# Autodesk Inventor assembly: OBG-Unterbau
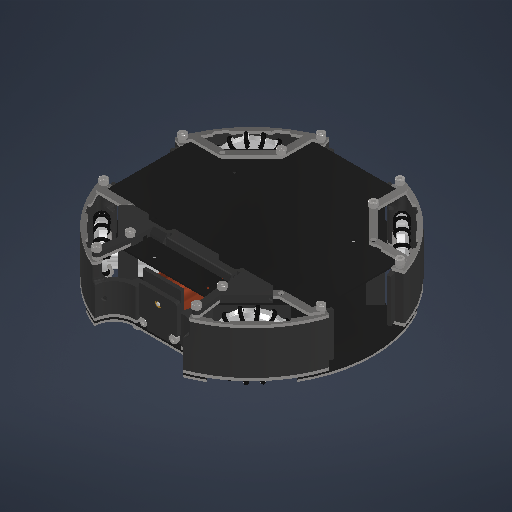
[picture p0: Inventor's stored thumbnail of the model, 512x512]
Saved by Autodesk Inventor 2025.2 (Build 292293000, 293)
## iProperties
Created: 2025-03-27
Part Number: OBG-Unterbau
Document SubType Name: Assembly
Designer: Faabs
Author: Faabs
## Documents named in this file (12)
- C:\Users\Faabs\Desktop\HBG v2023\OBG\Unterbau\OBG-Unterbau.iam
- C:\Users\Faabs\Desktop\HBG v2023\Platinen\Bodenplatine.ipt
- C:\Users\Faabs\Desktop\HBG v2023\UBG\Antrieb\UBG-Antrieb_VR.iam
- C:\Users\Faabs\Desktop\HBG v2023\UBG\Antrieb\UBG-Antrieb_VL.iam
- C:\Users\Faabs\Desktop\HBG v2023\UBG\Antrieb\UBG-Antrieb_HL.iam
- C:\Users\Faabs\Desktop\HBG v2023\UBG\Antrieb\UBG-Antrieb_HR.iam
- C:\Users\Faabs\Desktop\HBG v2023\UBG\Schuss\UBG-Schuss.iam
- C:\Users\Faabs\Desktop\HBG v2023\OBG\Unterbau\Bodenplatinenring.ipt
- C:\Users\Faabs\Desktop\HBG v2023\Platinen\Hauptplatine.ipt
- C:\Users\Faabs\Desktop\HBG v2023\UBG\Schutz\UBG-Schutz.iam
- C:\Users\Faabs\Desktop\HBG v2023\Verbindungselemente\DIN 912\DIN 912 - M3 x 0,5 x 6 x 4,75.ipt
- C:\Users\Faabs\Desktop\HBG v2023\OBG\Unterbau\Dribblerhalterung\Dribblerhalterung\Dribblerhalterung.ipt
## Components (28 placed, 11 different names)
1. UBG-Antrieb_VR:1 [sub-assembly] — Passend:2, Passend:3, Passend:16
2. UBG-Antrieb_VL:1 [sub-assembly] — Passend:4, Passend:5, Passend:15, Passend:20
3. UBG-Antrieb_HL:1 [sub-assembly] — Passend:6, Passend:7, Passend:8, Passend:22
4. UBG-Antrieb_HR:1 [sub-assembly] — Passend:9, Passend:10, Passend:11, Passend:21
5. UBG-Schuss:1 [sub-assembly] — Passend:12, Passend:13, Passend:14, Passend:15, Passend:16
6. UBG-Schutz:1 [sub-assembly] — Passend:23, Passend:24, Passend:25, Einfügen:1, Einfügen:2, Passend:26, Passend:27, Passend:28
7. Bodenplatine:1 — Passend:1, Fluchtend:1, Fluchtend:2, Passend:2, Passend:3, Passend:4, Passend:5, Passend:6, Passend:7, Passend:8, Passend:9, Passend:10, Passend:11, Passend:12, Passend:13, Passend:14, Passend:17, Passend:18, Passend:19, Passend:23, Passend:24, Passend:25
8. Hauptplatine:1 — Passend:20, Passend:21, Passend:22
9. Bodenplatinenring:1 — Passend:17, Passend:18, Passend:19, Einfügen:3, Einfügen:4, Einfügen:5, Einfügen:6, Einfügen:7, Einfügen:8, Einfügen:9, Einfügen:10, Einfügen:11, Einfügen:12, Einfügen:13, Einfügen:14
10. Dribblerhalterung:1 — Passend:26, Passend:27, Passend:28, Einfügen:15, Einfügen:16, Einfügen:17, Einfügen:18
11. DIN 912 - ersetzt durch DIN EN ISO 4762 M3 x 6:18 — Einfügen:17
12. DIN 912 - ersetzt durch DIN EN ISO 4762 M3 x 6:17 — Einfügen:18
13. DIN 912 - ersetzt durch DIN EN ISO 4762 M3 x 6:16 — Einfügen:15
14. DIN 912 - ersetzt durch DIN EN ISO 4762 M3 x 6:15 — Einfügen:16
15. DIN 912 - ersetzt durch DIN EN ISO 4762 M3 x 6:1 — Einfügen:1
16. DIN 912 - ersetzt durch DIN EN ISO 4762 M3 x 6:2 — Einfügen:2
17. DIN 912 - ersetzt durch DIN EN ISO 4762 M3 x 6:3 — Einfügen:5
18. DIN 912 - ersetzt durch DIN EN ISO 4762 M3 x 6:4 — Einfügen:6
19. DIN 912 - ersetzt durch DIN EN ISO 4762 M3 x 6:5 — Einfügen:3
20. DIN 912 - ersetzt durch DIN EN ISO 4762 M3 x 6:6 — Einfügen:4
21. DIN 912 - ersetzt durch DIN EN ISO 4762 M3 x 6:7 — Einfügen:14
22. DIN 912 - ersetzt durch DIN EN ISO 4762 M3 x 6:8 — Einfügen:13
23. DIN 912 - ersetzt durch DIN EN ISO 4762 M3 x 6:9 — Einfügen:12
24. DIN 912 - ersetzt durch DIN EN ISO 4762 M3 x 6:10 — Einfügen:11
25. DIN 912 - ersetzt durch DIN EN ISO 4762 M3 x 6:11 — Einfügen:10
26. DIN 912 - ersetzt durch DIN EN ISO 4762 M3 x 6:12 — Einfügen:9
27. DIN 912 - ersetzt durch DIN EN ISO 4762 M3 x 6:13 — Einfügen:8
28. DIN 912 - ersetzt durch DIN EN ISO 4762 M3 x 6:14 — Einfügen:7
## Relationships (48: Mate 28, Insert 18, Flush 2)
- Passend:1 [Mate]: Bodenplatine:1
- Fluchtend:1 [Flush]: Bodenplatine:1
- Fluchtend:2 [Flush]: Bodenplatine:1
- Passend:2 [Mate]: UBG-Antrieb_VR:1 ↔ Bodenplatine:1
- Passend:3 [Mate]: UBG-Antrieb_VR:1 ↔ Bodenplatine:1
- Passend:4 [Mate]: UBG-Antrieb_VL:1 ↔ Bodenplatine:1
- Passend:5 [Mate]: UBG-Antrieb_VL:1 ↔ Bodenplatine:1
- Passend:6 [Mate]: UBG-Antrieb_HL:1 ↔ Bodenplatine:1
- Passend:7 [Mate]: UBG-Antrieb_HL:1 ↔ Bodenplatine:1
- Passend:8 [Mate]: UBG-Antrieb_HL:1 ↔ Bodenplatine:1
- Passend:9 [Mate]: UBG-Antrieb_HR:1 ↔ Bodenplatine:1
- Passend:10 [Mate]: UBG-Antrieb_HR:1 ↔ Bodenplatine:1
- Passend:11 [Mate]: UBG-Antrieb_HR:1 ↔ Bodenplatine:1
- Passend:12 [Mate]: UBG-Schuss:1 ↔ Bodenplatine:1
- Passend:13 [Mate]: UBG-Schuss:1 ↔ Bodenplatine:1
- Passend:14 [Mate]: UBG-Schuss:1 ↔ Bodenplatine:1
- Passend:15 [Mate]: UBG-Antrieb_VL:1 ↔ UBG-Schuss:1
- Passend:16 [Mate]: UBG-Antrieb_VR:1 ↔ UBG-Schuss:1
- Passend:17 [Mate]: Bodenplatine:1 ↔ Bodenplatinenring:1
- Passend:18 [Mate]: Bodenplatine:1 ↔ Bodenplatinenring:1
- Passend:19 [Mate]: Bodenplatine:1 ↔ Bodenplatinenring:1
- Passend:20 [Mate]: UBG-Antrieb_VL:1 ↔ Hauptplatine:1
- Passend:21 [Mate]: UBG-Antrieb_HR:1 ↔ Hauptplatine:1
- Passend:22 [Mate]: UBG-Antrieb_HL:1 ↔ Hauptplatine:1
- Passend:23 [Mate]: UBG-Schutz:1 ↔ Bodenplatine:1
- Passend:24 [Mate]: UBG-Schutz:1 ↔ Bodenplatine:1
- Passend:25 [Mate]: UBG-Schutz:1 ↔ Bodenplatine:1
- Einfügen:1 [Insert]: UBG-Schutz:1 ↔ DIN 912 - ersetzt durch DIN EN ISO 4762 M3 x 6:1
- Einfügen:2 [Insert]: UBG-Schutz:1 ↔ DIN 912 - ersetzt durch DIN EN ISO 4762 M3 x 6:2
- Einfügen:3 [Insert]: Bodenplatinenring:1 ↔ DIN 912 - ersetzt durch DIN EN ISO 4762 M3 x 6:5
- Einfügen:4 [Insert]: Bodenplatinenring:1 ↔ DIN 912 - ersetzt durch DIN EN ISO 4762 M3 x 6:6
- Einfügen:5 [Insert]: Bodenplatinenring:1 ↔ DIN 912 - ersetzt durch DIN EN ISO 4762 M3 x 6:3
- Einfügen:6 [Insert]: Bodenplatinenring:1 ↔ DIN 912 - ersetzt durch DIN EN ISO 4762 M3 x 6:4
- Einfügen:7 [Insert]: Bodenplatinenring:1 ↔ DIN 912 - ersetzt durch DIN EN ISO 4762 M3 x 6:14
- Einfügen:8 [Insert]: Bodenplatinenring:1 ↔ DIN 912 - ersetzt durch DIN EN ISO 4762 M3 x 6:13
- Einfügen:9 [Insert]: Bodenplatinenring:1 ↔ DIN 912 - ersetzt durch DIN EN ISO 4762 M3 x 6:12
- Einfügen:10 [Insert]: Bodenplatinenring:1 ↔ DIN 912 - ersetzt durch DIN EN ISO 4762 M3 x 6:11
- Einfügen:11 [Insert]: Bodenplatinenring:1 ↔ DIN 912 - ersetzt durch DIN EN ISO 4762 M3 x 6:10
- Einfügen:12 [Insert]: Bodenplatinenring:1 ↔ DIN 912 - ersetzt durch DIN EN ISO 4762 M3 x 6:9
- Einfügen:13 [Insert]: Bodenplatinenring:1 ↔ DIN 912 - ersetzt durch DIN EN ISO 4762 M3 x 6:8
- Einfügen:14 [Insert]: Bodenplatinenring:1 ↔ DIN 912 - ersetzt durch DIN EN ISO 4762 M3 x 6:7
- Passend:26 [Mate]: UBG-Schutz:1 ↔ Dribblerhalterung:1
- Passend:27 [Mate]: UBG-Schutz:1 ↔ Dribblerhalterung:1
- Passend:28 [Mate]: UBG-Schutz:1 ↔ Dribblerhalterung:1
- Einfügen:15 [Insert]: Dribblerhalterung:1 ↔ DIN 912 - ersetzt durch DIN EN ISO 4762 M3 x 6:16
- Einfügen:16 [Insert]: Dribblerhalterung:1 ↔ DIN 912 - ersetzt durch DIN EN ISO 4762 M3 x 6:15
- Einfügen:17 [Insert]: Dribblerhalterung:1 ↔ DIN 912 - ersetzt durch DIN EN ISO 4762 M3 x 6:18
- Einfügen:18 [Insert]: Dribblerhalterung:1 ↔ DIN 912 - ersetzt durch DIN EN ISO 4762 M3 x 6:17
